# Autodesk Inventor assembly: Roue_moteur
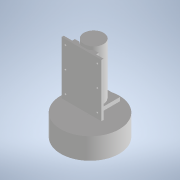
[picture p0: Inventor's stored thumbnail of the model, 180x180]
Saved by Autodesk Inventor 2020.1 (Build 241239000, 239)
## iProperties
Created: 2019-11-15
Part Number: Roue_moteur
Document SubType Name: Assembly
Designer: Admin
Author: Admin
## Documents named in this file (5)
- C:\Users\Admin\Desktop\Projet OrangeLab\Montage avec roue Crawler\Roue_moteur.iam
- C:\Users\Admin\Desktop\Projet OrangeLab\Montage avec roue Crawler\Adaptateur_axes.ipt
- C:\Users\Admin\Desktop\Projet OrangeLab\Montage avec roue Crawler\Moteur.ipt
- C:\Users\Admin\Desktop\Projet OrangeLab\Montage avec roue Crawler\Roue_Crawler.ipt
- C:\Users\Admin\Desktop\Projet OrangeLab\Montage avec roue Crawler\Support_moteur.ipt
## Components (4 placed, 4 different names)
1. Adaptateur_axes:1 — Mate:4, Mate:5, Mate:6, Mate:7
2. Moteur:1 — Mate:1, Mate:2, Mate:3, Mate:6, Mate:7
3. Roue_Crawler:1 — Mate:4, Mate:5
4. Support_moteur:1 — Mate:1, Mate:2, Mate:3
## Relationships (7: Mate 7)
- Mate:1: Moteur:1 ↔ Support_moteur:1
- Mate:2: Moteur:1 ↔ Support_moteur:1
- Mate:3: Moteur:1 ↔ Support_moteur:1
- Mate:4: Adaptateur_axes:1 ↔ Roue_Crawler:1
- Mate:5: Adaptateur_axes:1 ↔ Roue_Crawler:1
- Mate:6: Adaptateur_axes:1 ↔ Moteur:1
- Mate:7: Adaptateur_axes:1 ↔ Moteur:1
